# Autodesk Inventor assembly: electronics_assy
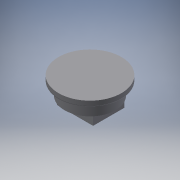
[picture p0: Inventor's stored thumbnail of the model, 180x180]
Saved by Autodesk Inventor 2017 (Build 210142000, 142)
## iProperties
Created: 2019-05-26
Part Number: electronics_assy
Document SubType Name: Assembly
Designer: Mitch
Author: Mitch
## Documents named in this file (4)
- E:\Youtube Channel\Pojects\Scammer Away\Mech\electronics_assy.iam
- E:\Youtube Channel\Pojects\Scammer Away\Mech\battery board.ipt
- E:\Youtube Channel\Pojects\Scammer Away\Mech\speaker.ipt
- E:\Youtube Channel\Pojects\Scammer Away\Mech\MP#.ipt
## Components (3 placed, 3 different names)
1. battery board:1 — Mate:1, Mate:2, Mate:3, Tangent:1
2. speaker:1 — Mate:1, Mate:2
3. MP#:1 — Mate:3, Tangent:1
## Relationships (4: Mate 3, Tangent 1)
- Mate:1: battery board:1 ↔ speaker:1
- Mate:2: battery board:1 ↔ speaker:1
- Mate:3: battery board:1 ↔ MP#:1
- Tangent:1 (-22.86 mm): battery board:1 ↔ MP#:1
